# Autodesk Inventor assembly: Right Door
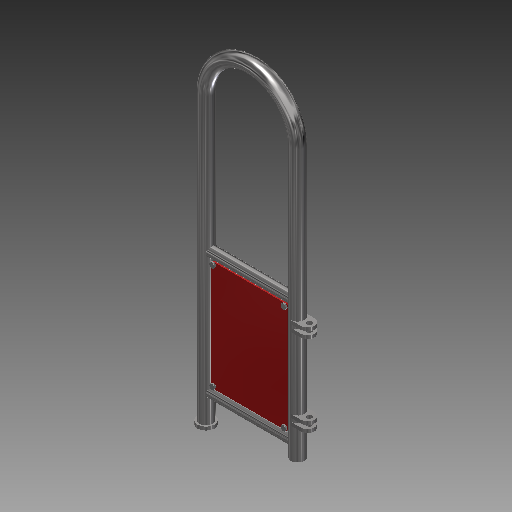
[picture p0: Inventor's stored thumbnail of the model, 512x512]
Saved by Autodesk Inventor 2018 (Build 220112000, 112)
## iProperties
Created: 2018-02-10
Part Number: Right Door
Document SubType Name: Assembly
Designer: Joey
Author: Joey
## Documents named in this file (5)
- M:\TPS\9th Grade\CADD 2017-2018\Current\Ferris Wheel Group Project\Group Project Week 3\Gondola\Right Door.iam
- M:\TPS\9th Grade\CADD 2017-2018\Current\Ferris Wheel Group Project\Group Project Week 3\Gondola\Door Frame.ipt
- M:\TPS\9th Grade\CADD 2017-2018\Current\Ferris Wheel Group Project\Group Project Week 3\Gondola\Door Plate.ipt
- M:\TPS\9th Grade\CADD 2017-2018\Current\Ferris Wheel Group Project\Group Project Week 3\Gondola\Door Plate Nut.ipt
- M:\TPS\9th Grade\CADD 2017-2018\Current\Ferris Wheel Group Project\Group Project Week 3\Gondola\Door Plate Screw.ipt
## Components (10 placed, 4 different names)
1. Door Frame:1 — Mate:1, Mate:2, Mate:3
2. Door Plate Nut:1 — Insert:5
3. Door Plate Screw:1 — Insert:7, Insert:12
4. Door Plate Nut:2 — Insert:7
5. Door Plate Screw:2 — Insert:8, Insert:11
6. Door Plate Nut:3 — Insert:8
7. Door Plate Screw:3 — Insert:5, Insert:10
8. Door Plate Nut:4 — Insert:6
9. Door Plate Screw:4 — Insert:6, Insert:9
10. Door Plate:1 — Mate:1, Mate:2, Mate:3, Insert:9, Insert:10, Insert:11, Insert:12
## Relationships (11: Insert 8, Mate 3)
- Insert:5: Door Plate Nut:1 ↔ Door Plate Screw:3
- Insert:6: Door Plate Nut:4 ↔ Door Plate Screw:4
- Insert:7: Door Plate Screw:1 ↔ Door Plate Nut:2
- Insert:8: Door Plate Screw:2 ↔ Door Plate Nut:3
- Mate:1: Door Frame:1 ↔ Door Plate:1
- Mate:2: Door Frame:1 ↔ Door Plate:1
- Mate:3: Door Frame:1 ↔ Door Plate:1
- Insert:9: Door Plate Screw:4 ↔ Door Plate:1
- Insert:10: Door Plate Screw:3 ↔ Door Plate:1
- Insert:11: Door Plate Screw:2 ↔ Door Plate:1
- Insert:12: Door Plate Screw:1 ↔ Door Plate:1
